# Autodesk Inventor assembly: Сборка_электр
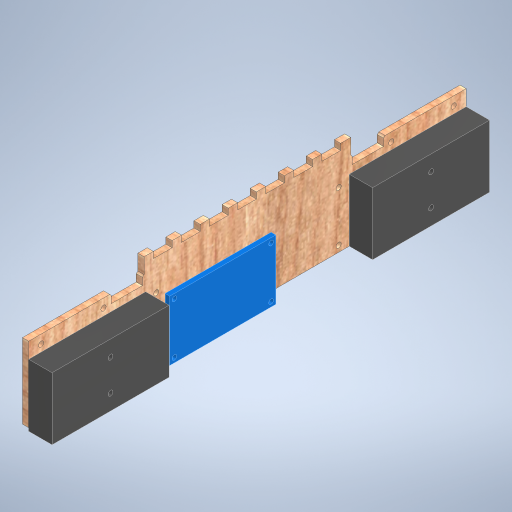
[picture p0: Inventor's stored thumbnail of the model, 512x512]
Saved by Autodesk Inventor 2023.1 (Build 271208000, 208)
## iProperties
Created: 2026-02-22
Part Number: Сборка_электр
Document SubType Name: Assembly
Designer: DELL
Author: DELL
## Documents named in this file (4)
- C:\Users\DELL\reposGitHub\VSOSH25-26\models\plotter\plotter_actual\Сборка_электр.iam
- C:\Users\DELL\reposGitHub\VSOSH25-26\models\plotter\plotter_actual\фанера_жлектроника_новая.ipt
- C:\Users\DELL\reposGitHub\VSOSH25-26\models\plotter\plotter_actual\холдер.ipt
- C:\Users\DELL\reposGitHub\VSOSH25-26\models\plotter\plotter_actual\inout\Понижающий_преобразователь_напряжения.ipt
## Components (4 placed, 3 different names)
1. фанера_жлектроника_новая:1 — Совмещение:1, Заподлицо:1, Совмещение:2, Заподлицо:2, Заподлицо:3, Заподлицо:4, Совмещение:3
2. холдер:1 — Заподлицо:1, Совмещение:2, Заподлицо:2
3. холдер:2 — Заподлицо:3, Заподлицо:4, Совмещение:3
4. Понижающий_преобразователь_напряжения:1
## Relationships (7: Flush 4, Mate 3)
- Совмещение:1 [Mate]: фанера_жлектроника_новая:1
- Заподлицо:1 [Flush]: фанера_жлектроника_новая:1 ↔ холдер:1
- Совмещение:2 [Mate]: фанера_жлектроника_новая:1 ↔ холдер:1
- Заподлицо:2 [Flush]: фанера_жлектроника_новая:1 ↔ холдер:1
- Заподлицо:3 [Flush]: фанера_жлектроника_новая:1 ↔ холдер:2
- Заподлицо:4 [Flush]: фанера_жлектроника_новая:1 ↔ холдер:2
- Совмещение:3 [Mate]: фанера_жлектроника_новая:1 ↔ холдер:2
